# Autodesk Inventor assembly: 217-2000
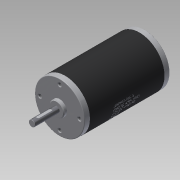
[picture p0: Inventor's stored thumbnail of the model, 180x180]
Saved by Autodesk Inventor 2020.1 (Build 241239000, 239)
## iProperties
Category: VEXpro Motor Box
Company: Autodesk, Inc.
Document SubType Name: Assembly
Created: 2019-11-13
Project: FIRST
Part Number: 217-2000
Description: CIM Motor
Catalog Web Link: https://www.vexrobotics.com/217-2000.html
Vendor: IFI
Control State: 0
Master: False
Checked Out: False
Shininess: 64.0
Length Units: 11272
Angle Units: 11279
Time Units: 11290
Mass Units: 11286
Length Display Precision: 3
Angle Display Precision: 2
Compacted: True
Density: 0.0
Volumn: 0.0
Area: 0.0
PropertySet Name: Model Information
Title: CIM Motor
Author: Autodesk, Inc.
Keywords: Separate Tote
## Documents named in this file (3)
- D:\FIRST 2020\FRC 2020\FRC KOP 2020\Inventor\217-2000.iam
- D:\FIRST 2020\FRC 2020\FRC KOP 2020\Inventor\Parts\FR801-001_CIM Motor Body.ipt
- D:\FIRST 2020\FRC 2020\FRC KOP 2020\Inventor\Parts\FR801-001_CIM Motor Machine Screw.ipt
## Components (3 placed, 2 different names)
1. FR801-001_CIM Motor Body:1 — Insert:1, Insert:2
2. FR801-001_CIM Motor Machine Screw:1 — Insert:1
3. FR801-001_CIM Motor Machine Screw:2 — Insert:2
## Relationships (2: Insert 2)
- Insert:1: FR801-001_CIM Motor Body:1 ↔ FR801-001_CIM Motor Machine Screw:1
- Insert:2: FR801-001_CIM Motor Body:1 ↔ FR801-001_CIM Motor Machine Screw:2
